# Autodesk Inventor assembly: MK4 Billet Wheel Assembly
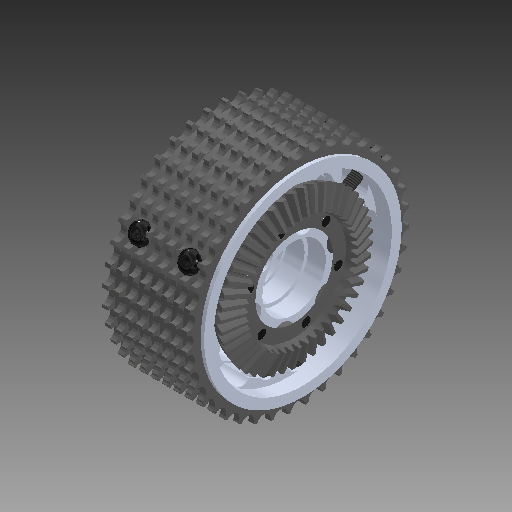
[picture p0: Inventor's stored thumbnail of the model, 512x512]
Saved by Autodesk Inventor 2025 (Build 290162010, 162A)
## iProperties
Created: 2024-07-13
Part Number: MK4 Billet Wheel Assembly
Document SubType Name: Assembly
Designer: rohan
Author: rohan
Revision Number: ANY
## Documents named in this file (7)
- D:\ultimate-hecker\Computer-Aided-Design\FRC-Offseason-Design-Training\Parts Library\Drivetrains\Swerve Modules\MK4\MK4 Billet Wheel Assembly.iam
- D:\ultimate-hecker\Computer-Aided-Design\FRC-Offseason-Design-Training\Parts Library\Drivetrains\Swerve Modules\SDS MK4 Swerve Module, Falcons\Wheel, SDS, Nitrile Tread, 4in X 1.5in, Bearing Bore.ipt
- D:\ultimate-hecker\Computer-Aided-Design\FRC-Offseason-Design-Training\Parts Library\Power Transfer\Gears (Bevel)\Bevel Gear (4515).ipt
- D:\ultimate-hecker\Computer-Aided-Design\FRC-Offseason-Design-Training\Parts Library\Hardware\Fasteners\Machine Screws\10-32 UNFx0.75 Button Head Cap Screw.ipt
- D:\ultimate-hecker\Computer-Aided-Design\FRC-Offseason-Design-Training\Parts Library\Hardware\Fasteners\Machine Screws.ipt
- D:\ultimate-hecker\Computer-Aided-Design\FRC-Offseason-Design-Training\Parts Library\Hardware\Fasteners\Machine Screws\10-32 UNFx0.5 Button Head Cap Screw.ipt
- D:\ultimate-hecker\Computer-Aided-Design\FRC-Offseason-Design-Training\Parts Library\Wheels\Billet Wheels\Black NitrileThread 4in X 1.5in.ipt
## Components (17 placed, 17 different names)
1. Wheel, SDS, Nitrile Tread, 4in X 1.5in, Bearing Bore_81 — Insert:1, Insert:2, Insert:3, Insert:4, Insert:5, Insert:6, Insert:7, Insert:8, Insert:9, Symmetry:1
2. Tread, Blue Nitrile 4in X 1.5in_82 — Insert:9, Insert:10, Insert:11, Insert:12, Insert:13, Insert:14, Insert:15, Insert:16, Insert:17, Symmetry:1, Tangent:1
3. Bevel Gear, 4515_83 — Insert:7, Insert:8
4. Screw, 10-32 X .75, Button, 91255A269_91255A269_84 — Insert:5
5. Screw, 10-32 X .75, Button, 91255A269_91255A269_85 — Insert:4
6. Screw, 10-32 X .75, Button, 91255A269_91255A269_86 — Insert:6
7. Screw, 10-32 X .75, Button, 91255A269_91255A269_87 — Insert:3
8. Screw, 10-32 X .75, Button, 91255A269_91255A269_88 — Insert:2
9. Screw, 10-32 X .75, Button, 91255A269_91255A269_89 — Insert:1
10. Screw, 10-32 X .5, Button, 97763A232_97763A232_90 — Insert:17
11. Screw, 10-32 X .5, Button, 97763A232_97763A232_91 — Insert:16
12. Screw, 10-32 X .5, Button, 97763A232_97763A232_92 — Insert:15
13. Screw, 10-32 X .5, Button, 97763A232_97763A232_93 — Insert:14
14. Screw, 10-32 X .5, Button, 97763A232_97763A232_94 — Insert:10
15. Screw, 10-32 X .5, Button, 97763A232_97763A232_95 — Insert:11
16. Screw, 10-32 X .5, Button, 97763A232_97763A232_96 — Insert:13
17. Screw, 10-32 X .5, Button, 97763A232_97763A232_97 — Insert:12
## Relationships (19: Insert 17, Symmetry 1, Tangent 1)
- Insert:1: Wheel, SDS, Nitrile Tread, 4in X 1.5in, Bearing Bore_81 ↔ Screw, 10-32 X .75, Button, 91255A269_91255A269_89
- Insert:2: Wheel, SDS, Nitrile Tread, 4in X 1.5in, Bearing Bore_81 ↔ Screw, 10-32 X .75, Button, 91255A269_91255A269_88
- Insert:3: Wheel, SDS, Nitrile Tread, 4in X 1.5in, Bearing Bore_81 ↔ Screw, 10-32 X .75, Button, 91255A269_91255A269_87
- Insert:4: Wheel, SDS, Nitrile Tread, 4in X 1.5in, Bearing Bore_81 ↔ Screw, 10-32 X .75, Button, 91255A269_91255A269_85
- Insert:5: Wheel, SDS, Nitrile Tread, 4in X 1.5in, Bearing Bore_81 ↔ Screw, 10-32 X .75, Button, 91255A269_91255A269_84
- Insert:6: Wheel, SDS, Nitrile Tread, 4in X 1.5in, Bearing Bore_81 ↔ Screw, 10-32 X .75, Button, 91255A269_91255A269_86
- Insert:7: Wheel, SDS, Nitrile Tread, 4in X 1.5in, Bearing Bore_81 ↔ Bevel Gear, 4515_83
- Insert:8: Wheel, SDS, Nitrile Tread, 4in X 1.5in, Bearing Bore_81 ↔ Bevel Gear, 4515_83
- Insert:9: Wheel, SDS, Nitrile Tread, 4in X 1.5in, Bearing Bore_81 ↔ Tread, Blue Nitrile 4in X 1.5in_82
- Insert:10: Tread, Blue Nitrile 4in X 1.5in_82 ↔ Screw, 10-32 X .5, Button, 97763A232_97763A232_94
- Insert:11: Tread, Blue Nitrile 4in X 1.5in_82 ↔ Screw, 10-32 X .5, Button, 97763A232_97763A232_95
- Insert:12: Tread, Blue Nitrile 4in X 1.5in_82 ↔ Screw, 10-32 X .5, Button, 97763A232_97763A232_97
- Insert:13: Tread, Blue Nitrile 4in X 1.5in_82 ↔ Screw, 10-32 X .5, Button, 97763A232_97763A232_96
- Insert:14: Tread, Blue Nitrile 4in X 1.5in_82 ↔ Screw, 10-32 X .5, Button, 97763A232_97763A232_93
- Insert:15: Tread, Blue Nitrile 4in X 1.5in_82 ↔ Screw, 10-32 X .5, Button, 97763A232_97763A232_92
- Insert:16: Tread, Blue Nitrile 4in X 1.5in_82 ↔ Screw, 10-32 X .5, Button, 97763A232_97763A232_91
- Insert:17: Tread, Blue Nitrile 4in X 1.5in_82 ↔ Screw, 10-32 X .5, Button, 97763A232_97763A232_90
- Symmetry:1: Wheel, SDS, Nitrile Tread, 4in X 1.5in, Bearing Bore_81 ↔ Tread, Blue Nitrile 4in X 1.5in_82
- Tangent:1: Tread, Blue Nitrile 4in X 1.5in_82
